# Autodesk Inventor assembly: SUBReserviorPiston
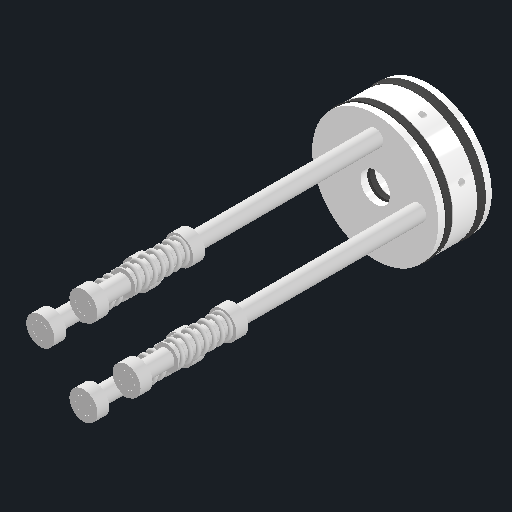
[picture p0: Inventor's stored thumbnail of the model, 512x512]
Saved by Autodesk Inventor 2024 (Build 280153000, 153)
## iProperties
Created: 2025-02-07
Part Number: SUBReserviorPiston
Document SubType Name: Assembly
Designer: Tommy Rohmann
Author: Tommy Rohmann
## Documents named in this file (6)
- C:\Users\Tommy Rohmann\OneDrive\Projects\Microgravity-Press-Washing-Machine\System Design and Documentation\Inventor Design Project\SUBReserviorPiston.iam
- C:\Users\Tommy Rohmann\OneDrive\Projects\Microgravity-Press-Washing-Machine\System Design and Documentation\Inventor Design Project\LAYOUT.ipt
- C:\Users\Tommy Rohmann\OneDrive\Projects\Microgravity-Press-Washing-Machine\System Design and Documentation\Inventor Design Project\ReserviorPiston.ipt
- C:\Users\Tommy Rohmann\OneDrive\Projects\Microgravity-Press-Washing-Machine\System Design and Documentation\Inventor Design Project\DynamicPistonSeal.ipt
- C:\Users\Tommy Rohmann\OneDrive\Projects\Microgravity-Press-Washing-Machine\System Design and Documentation\Inventor Design Project\DynamicRodSeal.ipt
- C:\Users\Tommy Rohmann\OneDrive\Projects\Microgravity-Press-Washing-Machine\System Design and Documentation\Inventor Design Project\SUBReserviorPistonRod.iam
## Components (10 placed, 5 different names)
1. LAYOUT:1
2. ReserviorPiston:1 — Mate:5, Mate:6, Mate:9, Mate:10, Mate:11, Mate:12, Mate:13, Mate:14, Mate:15, Mate:16, Mate:17, Mate:18, Mate:19, Mate:20, Mate:21, Mate:22, Mate:23, Mate:24
3. DynamicPistonSeal:1 — Mate:14, Mate:15
4. DynamicRodSeal:1 — Mate:11, Mate:16
5. DynamicPistonSeal:2 — Mate:9, Mate:10
6. DynamicRodSeal:2 — Mate:12, Mate:13
7. SUBReserviorPistonRod:1 [sub-assembly] — Mate:17, Mate:18
8. SUBReserviorPistonRod:2 [sub-assembly] — Mate:21, Mate:22
9. SUBReserviorPistonRod:3 [sub-assembly] — Mate:20, Mate:23
10. SUBReserviorPistonRod:4 [sub-assembly] — Mate:19, Mate:24
## Relationships (24: Mate 22, Composite 1, Angle 1)
- [Composite]: LAYOUT:1 ↔ ReserviorPiston:1
- Mate:3
- Mate:4
- Mate:5: ReserviorPiston:1
- Mate:6: ReserviorPiston:1
- Mate:7
- Mate:8
- Angle:1 (0 deg)
- Mate:9: ReserviorPiston:1 ↔ DynamicPistonSeal:2
- Mate:10: ReserviorPiston:1 ↔ DynamicPistonSeal:2
- Mate:11: ReserviorPiston:1 ↔ DynamicRodSeal:1
- Mate:12: ReserviorPiston:1 ↔ DynamicRodSeal:2
- Mate:13: ReserviorPiston:1 ↔ DynamicRodSeal:2
- Mate:14: ReserviorPiston:1 ↔ DynamicPistonSeal:1
- Mate:15: ReserviorPiston:1 ↔ DynamicPistonSeal:1
- Mate:16: ReserviorPiston:1 ↔ DynamicRodSeal:1
- Mate:17: ReserviorPiston:1 ↔ SUBReserviorPistonRod:1
- Mate:18: ReserviorPiston:1 ↔ SUBReserviorPistonRod:1
- Mate:19: ReserviorPiston:1 ↔ SUBReserviorPistonRod:4
- Mate:20: ReserviorPiston:1 ↔ SUBReserviorPistonRod:3
- Mate:21: ReserviorPiston:1 ↔ SUBReserviorPistonRod:2
- Mate:22: ReserviorPiston:1 ↔ SUBReserviorPistonRod:2
- Mate:23: ReserviorPiston:1 ↔ SUBReserviorPistonRod:3
- Mate:24: ReserviorPiston:1 ↔ SUBReserviorPistonRod:4
